# Autodesk Inventor assembly: Shock Cartridge
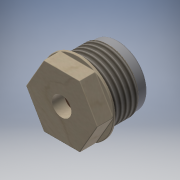
[picture p0: Inventor's stored thumbnail of the model, 180x180]
Saved by Autodesk Inventor 2019 (Build 230136000, 136)
## iProperties
Created: 2019-12-02
Part Number: Shock Cartridge
Document SubType Name: Assembly
Designer: Jopa
Author: Jopa
## Documents named in this file (5)
- C:\Users\Jopa\Desktop\Suspension\Shock Cartridge.iam
- C:\Users\Jopa\Desktop\Suspension\Shock Cartridge.ipt
- C:\Users\Jopa\Desktop\Suspension\O-Ring.ipt
- C:\Users\Jopa\Desktop\Suspension\Shock Cartridge Spacer.ipt
- C:\Users\Jopa\Desktop\Suspension\Shock Cartridge Cover.ipt
## Components (5 placed, 4 different names)
1. Shock Cartridge:1 — Mate:1, Mate:2, Mate:3, Mate:4, Mate:5, Mate:6
2. O-Ring:1 — Mate:1, Mate:2, Flush:1
3. Shock Cartridge Spacer:1 — Mate:3, Flush:1, Flush:2
4. Shock Cartridge Cover:1 — Mate:5, Mate:6
5. O-Ring:2 — Mate:4, Flush:2
## Relationships (8: Mate 6, Flush 2)
- Mate:1: Shock Cartridge:1 ↔ O-Ring:1
- Mate:2: Shock Cartridge:1 ↔ O-Ring:1
- Mate:3: Shock Cartridge:1 ↔ Shock Cartridge Spacer:1
- Flush:1: O-Ring:1 ↔ Shock Cartridge Spacer:1
- Mate:4: Shock Cartridge:1 ↔ O-Ring:2
- Flush:2: Shock Cartridge Spacer:1 ↔ O-Ring:2
- Mate:5: Shock Cartridge:1 ↔ Shock Cartridge Cover:1
- Mate:6: Shock Cartridge:1 ↔ Shock Cartridge Cover:1
